# Autodesk Inventor assembly: A_Wing_MIR
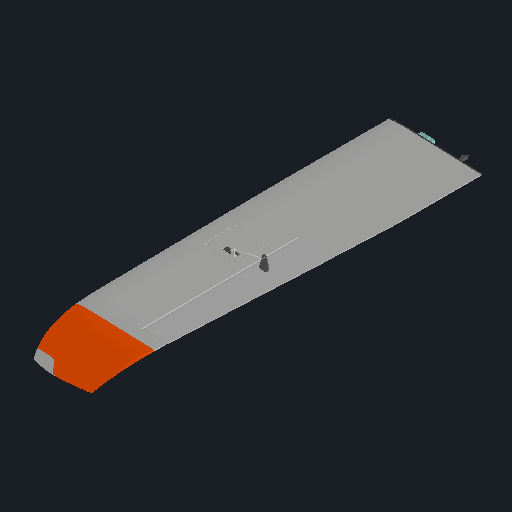
[picture p0: Inventor's stored thumbnail of the model, 512x512]
Saved by Autodesk Inventor 2026 (Build 300175000, 175)
## iProperties
Created: 2025-09-10
Part Number: A_Wing_MIR
Document SubType Name: Assembly
Designer: FAL
Author: FAL
## Documents named in this file (17)
- C:\Users\FAL\Projekte\Git\AIRBERT\CAD\Wing\mirror\A_Wing_MIR.iam
- C:\Users\FAL\Projekte\Git\AIRBERT\CAD\Wing\mirror\P_Wing_mid_servolink_MIR.ipt
- C:\Users\FAL\Projekte\Git\AIRBERT\CAD\Wing\mirror\P_Wing_inner_MIR.ipt
- C:\Users\FAL\Projekte\Git\AIRBERT\CAD\Wing\mirror\P_Wing_mid_MIR.ipt
- C:\Users\FAL\Projekte\Git\AIRBERT\CAD\Wing\mirror\P_Wing_mid_servocap_MIR.ipt
- C:\Users\FAL\Projekte\Git\AIRBERT\CAD\Wing\mirror\P_Wing_Mountingplate_MIR.ipt
- C:\Users\FAL\Projekte\Git\AIRBERT\CAD\Wing\mirror\P_Wing_winglet_MIR.ipt
- C:\Users\FAL\Projekte\Git\AIRBERT\CAD\Wing\mirror\P_Wing_winglet_LEDcap_MIR.ipt
- C:\Users\FAL\Projekte\Git\AIRBERT\CAD\Wing\mirror\P_Wing_aileron_MIR.ipt
- C:\Users\FAL\Projekte\Git\AIRBERT\CAD\Wing\mirror\P_Wing_aileron_lever_MIR.ipt
- C:\Users\FAL\Projekte\Git\AIRBERT\CAD\Wing\mirror\P_Wing_Mountingplate_pin_MIR.ipt
- C:\Users\FAL\Projekte\Git\AIRBERT\CAD\Wing\mirror\P_Wing_inner_add_MIR.ipt
- C:\Users\FAL\Projekte\Git\AIRBERT\CAD\Wing\mirror\P_JX9_F_ref_MIR.ipt
- C:\Users\FAL\Projekte\Git\AIRBERT\CAD\Wing\mirror\P_LED_5_MIR.ipt
- C:\Users\FAL\Projekte\Git\AIRBERT\CAD\Wing\mirror\P_Servo_SIMPROP_MIR.ipt
- C:\Users\FAL\Projekte\Git\AIRBERT\CAD\Wing\mirror\P_Servo_SIMPROP_lever_MIR.ipt
- C:\Users\FAL\Projekte\Git\AIRBERT\CAD\Wing\P_Wing.ipt
## Components (16 placed, 16 different names)
1. P_Wing_mid_servolink_MIR:1 — Tangential:1, Passend:19, Passend:18
2. P_Wing_inner_MIR:1 — Fluchtend:3, Fluchtend:2, Fluchtend:1, Passend:11, Passend:10, Passend:9, Passend:24, Passend:23
3. P_Wing_mid_MIR:1 — Fluchtend:6, Fluchtend:5, Fluchtend:4, Passend:26
4. P_Wing_mid_servocap_MIR:1 — Fluchtend:9, Fluchtend:8, Fluchtend:7
5. P_Wing_Mountingplate_MIR:1 — Fluchtend:12, Fluchtend:11, Fluchtend:10, Fluchtend:24, Passend:21, Passend:20, Passend:25, Passend:27
6. P_Wing_winglet_MIR:1 — Fluchtend:15, Fluchtend:14, Fluchtend:13
7. P_Wing_winglet_LEDcap_MIR:1 — Fluchtend:18, Fluchtend:17, Fluchtend:16, Passend:12, Passend:8
8. P_Wing_aileron_MIR:1 — Passend:26, Passend:15, Passend:14, Passend:13
9. P_Wing_aileron_lever_MIR:1 — Tangential:1, Passend:15, Passend:14, Passend:13
10. P_Wing_Mountingplate_pin_MIR:1 — Passend:25, Passend:24, Passend:23
11. P_Wing_inner_add_MIR:1 — Passend:27, Fluchtend:27, Fluchtend:26, Fluchtend:25
12. P_JX9_F_ref_MIR:1 — Fluchtend:24, Passend:21, Passend:20
13. P_LED_5_MIR:1 — Passend:12, Passend:8
14. P_Servo_SIMPROP_MIR:1 — Passend:11, Passend:10, Passend:9, Passend:6, Passend:5
15. P_Servo_SIMPROP_lever_MIR:1 — Passend:19, Passend:18, Passend:6, Passend:5
16. P_Wing:1
## Relationships (42: Flush 22, Mate 19, Tangent 1)
- Fluchtend:3 [Flush]: P_Wing_inner_MIR:1
- Fluchtend:2 [Flush]: P_Wing_inner_MIR:1
- Fluchtend:1 [Flush]: P_Wing_inner_MIR:1
- Fluchtend:6 [Flush]: P_Wing_mid_MIR:1
- Fluchtend:5 [Flush]: P_Wing_mid_MIR:1
- Fluchtend:4 [Flush]: P_Wing_mid_MIR:1
- Fluchtend:9 [Flush]: P_Wing_mid_servocap_MIR:1
- Fluchtend:8 [Flush]: P_Wing_mid_servocap_MIR:1
- Fluchtend:7 [Flush]: P_Wing_mid_servocap_MIR:1
- Tangential:1: P_Wing_mid_servolink_MIR:1 ↔ P_Wing_aileron_lever_MIR:1
- Fluchtend:12 [Flush]: P_Wing_Mountingplate_MIR:1
- Fluchtend:11 [Flush]: P_Wing_Mountingplate_MIR:1
- Fluchtend:10 [Flush]: P_Wing_Mountingplate_MIR:1
- Fluchtend:15 [Flush]: P_Wing_winglet_MIR:1
- Fluchtend:14 [Flush]: P_Wing_winglet_MIR:1
- Fluchtend:13 [Flush]: P_Wing_winglet_MIR:1
- Fluchtend:18 [Flush]: P_Wing_winglet_LEDcap_MIR:1
- Fluchtend:17 [Flush]: P_Wing_winglet_LEDcap_MIR:1
- Fluchtend:16 [Flush]: P_Wing_winglet_LEDcap_MIR:1
- Passend:26 [Mate]: P_Wing_mid_MIR:1 ↔ P_Wing_aileron_MIR:1
- Passend:15 [Mate] (0.2525 mm): P_Wing_aileron_MIR:1 ↔ P_Wing_aileron_lever_MIR:1
- Passend:14 [Mate] (0.25 mm): P_Wing_aileron_MIR:1 ↔ P_Wing_aileron_lever_MIR:1
- Passend:13 [Mate]: P_Wing_aileron_MIR:1 ↔ P_Wing_aileron_lever_MIR:1
- Fluchtend:24 [Flush]: P_Wing_Mountingplate_MIR:1 ↔ P_JX9_F_ref_MIR:1
- Passend:21 [Mate] (1.5 mm): P_Wing_Mountingplate_MIR:1 ↔ P_JX9_F_ref_MIR:1
- Passend:20 [Mate] (0.5 mm): P_Wing_Mountingplate_MIR:1 ↔ P_JX9_F_ref_MIR:1
- Passend:12 [Mate]: P_Wing_winglet_LEDcap_MIR:1 ↔ P_LED_5_MIR:1
- Passend:8 [Mate]: P_Wing_winglet_LEDcap_MIR:1 ↔ P_LED_5_MIR:1
- Passend:11 [Mate]: P_Wing_inner_MIR:1 ↔ P_Servo_SIMPROP_MIR:1
- Passend:10 [Mate]: P_Wing_inner_MIR:1 ↔ P_Servo_SIMPROP_MIR:1
- Passend:9 [Mate]: P_Wing_inner_MIR:1 ↔ P_Servo_SIMPROP_MIR:1
- Passend:19 [Mate]: P_Wing_mid_servolink_MIR:1 ↔ P_Servo_SIMPROP_lever_MIR:1
- Passend:18 [Mate]: P_Wing_mid_servolink_MIR:1 ↔ P_Servo_SIMPROP_lever_MIR:1
- Passend:6 [Mate]: P_Servo_SIMPROP_MIR:1 ↔ P_Servo_SIMPROP_lever_MIR:1
- Passend:5 [Mate]: P_Servo_SIMPROP_MIR:1 ↔ P_Servo_SIMPROP_lever_MIR:1
- Passend:25 [Mate] (7.5 mm): P_Wing_Mountingplate_MIR:1 ↔ P_Wing_Mountingplate_pin_MIR:1
- Passend:24 [Mate] (0.1 mm): P_Wing_inner_MIR:1 ↔ P_Wing_Mountingplate_pin_MIR:1
- Passend:23 [Mate] (0.1 mm): P_Wing_inner_MIR:1 ↔ P_Wing_Mountingplate_pin_MIR:1
- Passend:27 [Mate]: P_Wing_Mountingplate_MIR:1 ↔ P_Wing_inner_add_MIR:1
- Fluchtend:27 [Flush]: P_Wing_inner_add_MIR:1
- Fluchtend:26 [Flush]: P_Wing_inner_add_MIR:1
- Fluchtend:25 [Flush]: P_Wing_inner_add_MIR:1
